# Autodesk Inventor assembly: Swerve-Drivetrain-2
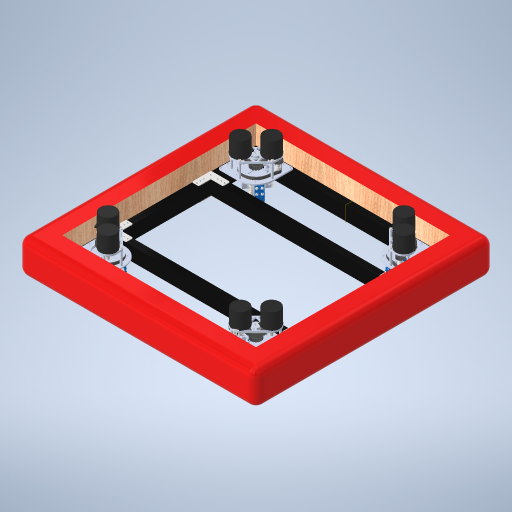
[picture p0: Inventor's stored thumbnail of the model, 512x512]
Saved by Autodesk Inventor 2024.2 (Build 282272000, 272)
## iProperties
Created: 2024-01-06
Part Number: Swerve-Drivetrain-2
Document SubType Name: Assembly
Designer: rohan
Author: rohan
## Documents named in this file (8)
- C:\Users\rohan\OneDrive - Hillsborough County Public Schools\Robotics\FIRST-Robotics-Competition\Crescendo\Minotaur-Crescendo-Robot\Swerve-Drivetrain-2.iam
- C:\Users\rohan\OneDrive - Hillsborough County Public Schools\Robotics\FIRST-Robotics-Competition\Crescendo\Minotaur-Crescendo-Robot\Motion\Swerve-Modules\MK3-Swerve-Module-Falcons-&-Neos.iam
- C:\Users\rohan\OneDrive - Hillsborough County Public Schools\Robotics\FIRST-Robotics-Competition\Crescendo\Minotaur-Crescendo-Robot\Structure\MAXTube\2024-100-002-Front-Back-Extrusions.ipt
- C:\Users\rohan\OneDrive - Hillsborough County Public Schools\Robotics\FIRST-Robotics-Competition\Crescendo\Minotaur-Crescendo-Robot\Structure\MAXTube\2024-100-001-Left-Right-Extrusions.ipt
- C:\Users\rohan\OneDrive - Hillsborough County Public Schools\Robotics\FIRST-Robotics-Competition\Crescendo\Minotaur-Crescendo-Robot\Structure\MAXTube\2024-100-003-Middle-Extrusions.ipt
- C:\Users\rohan\OneDrive - Hillsborough County Public Schools\Robotics\FIRST-Robotics-Competition\Crescendo\Minotaur-Crescendo-Robot\Structure\Gussets\90-Degree-Sharp-Gusset.ipt
- C:\Users\rohan\OneDrive - Hillsborough County Public Schools\Robotics\FIRST-Robotics-Competition\Crescendo\Minotaur-Crescendo-Robot\Structure\Gussets\THRIFYBOT-L-Gusset.ipt
- C:\Users\rohan\OneDrive - Hillsborough County Public Schools\Robotics\FIRST-Robotics-Competition\Crescendo\Minotaur-Crescendo-Robot\Bumpers.ipt
## Components (23 placed, 7 different names)
1. MK3-Swerve-Module-Falcons-&-Neos:1 [sub-assembly] — Mate:10, Mate:56, Mate:57
2. MK3-Swerve-Module-Falcons-&-Neos:2 [sub-assembly] — Mate:7, Mate:9, Mate:20
3. MK3-Swerve-Module-Falcons-&-Neos:3 [sub-assembly] — Mate:4, Mate:16, Tangent:1, Mate:52, Mate:53
4. MK3-Swerve-Module-Falcons-&-Neos:4 [sub-assembly] — Mate:1, Mate:2, Mate:3, Mate:14
5. 2024-100-002-Front-Back-Extrusions:1 — Mate:7, Mate:9, Mate:10, Mate:17, Flush:3, Flush:4, Mate:18, Flush:5, Mate:19, Flush:6, Symmetry:2, Mate:20, Mate:42, Mate:48, Mate:49, Mate:54, Mate:57, Flush:12, Flush:18
6. 2024-100-002-Front-Back-Extrusions:2 — Mate:1, Mate:2, Mate:3, Mate:4, Mate:13, Flush:1, Mate:15, Flush:2, Symmetry:2, Mate:40, Mate:41, Mate:44, Mate:45, Mate:46, Mate:47, Mate:52, Mate:53, Flush:20, Mate:65, Mate:66
7. 2024-100-001-Left-Right-Extrusions:1 — Mate:13, Mate:14, Flush:1, Symmetry:1, Mate:43
8. 2024-100-001-Left-Right-Extrusions:2 — Mate:15, Mate:16, Flush:2, Mate:17, Flush:3, Flush:4, Symmetry:1, Mate:55, Mate:56, Mate:67
9. 2024-100-003-Middle-Extrusions:1 — Mate:19, Flush:6, Symmetry:3, Mate:21, Mate:60, Flush:11, Flush:21
10. 2024-100-003-Middle-Extrusions:2 — Mate:18, Flush:5, Symmetry:3, Mate:21, Mate:61, Flush:13, Mate:64, Flush:19
11. 90-Degree-Sharp-Gusset:1 — Mate:42, Mate:54, Mate:55
12. 90-Degree-Sharp-Gusset:2 — Mate:43, Mate:48, Mate:49
13. 90-Degree-Sharp-Gusset:3 — Mate:41, Mate:44, Mate:45
14. 90-Degree-Sharp-Gusset:4 — Mate:40, Mate:46, Mate:47
15. THRIFYBOT-L-Gusset:1 — Mate:58, Flush:7, Flush:8
16. THRIFYBOT-L-Gusset:2 — Mate:58, Flush:7, Flush:8, Mate:60, Flush:11, Flush:12
17. THRIFYBOT-L-Gusset:3 — Mate:61
18. THRIFYBOT-L-Gusset:4 — Flush:13, Flush:18
19. THRIFYBOT-L-Gusset:5
20. THRIFYBOT-L-Gusset:6 — Mate:65, Flush:21
21. THRIFYBOT-L-Gusset:7
22. THRIFYBOT-L-Gusset:8 — Mate:64, Flush:19, Flush:20
23. Bumpers:1 — Mate:66, Mate:67, Mate:68
## Relationships (68: Mate 43, Flush 21, Symmetry 3, Tangent 1)
- Mate:1: MK3-Swerve-Module-Falcons-&-Neos:4 ↔ 2024-100-002-Front-Back-Extrusions:2
- Mate:2: MK3-Swerve-Module-Falcons-&-Neos:4 ↔ 2024-100-002-Front-Back-Extrusions:2
- Mate:3: MK3-Swerve-Module-Falcons-&-Neos:4 ↔ 2024-100-002-Front-Back-Extrusions:2
- Mate:4: MK3-Swerve-Module-Falcons-&-Neos:3 ↔ 2024-100-002-Front-Back-Extrusions:2
- Mate:7: MK3-Swerve-Module-Falcons-&-Neos:2 ↔ 2024-100-002-Front-Back-Extrusions:1
- Mate:9: MK3-Swerve-Module-Falcons-&-Neos:2 ↔ 2024-100-002-Front-Back-Extrusions:1
- Mate:10: MK3-Swerve-Module-Falcons-&-Neos:1 ↔ 2024-100-002-Front-Back-Extrusions:1
- Mate:13: 2024-100-002-Front-Back-Extrusions:2 ↔ 2024-100-001-Left-Right-Extrusions:1
- Mate:14: MK3-Swerve-Module-Falcons-&-Neos:4 ↔ 2024-100-001-Left-Right-Extrusions:1
- Flush:1: 2024-100-002-Front-Back-Extrusions:2 ↔ 2024-100-001-Left-Right-Extrusions:1
- Mate:15: 2024-100-002-Front-Back-Extrusions:2 ↔ 2024-100-001-Left-Right-Extrusions:2
- Mate:16: MK3-Swerve-Module-Falcons-&-Neos:3 ↔ 2024-100-001-Left-Right-Extrusions:2
- Flush:2: 2024-100-002-Front-Back-Extrusions:2 ↔ 2024-100-001-Left-Right-Extrusions:2
- Mate:17: 2024-100-002-Front-Back-Extrusions:1 ↔ 2024-100-001-Left-Right-Extrusions:2
- Flush:3: 2024-100-002-Front-Back-Extrusions:1 ↔ 2024-100-001-Left-Right-Extrusions:2
- Flush:4: 2024-100-002-Front-Back-Extrusions:1 ↔ 2024-100-001-Left-Right-Extrusions:2
- Mate:18: 2024-100-002-Front-Back-Extrusions:1 ↔ 2024-100-003-Middle-Extrusions:2
- Flush:5: 2024-100-002-Front-Back-Extrusions:1 ↔ 2024-100-003-Middle-Extrusions:2
- Mate:19: 2024-100-002-Front-Back-Extrusions:1 ↔ 2024-100-003-Middle-Extrusions:1
- Flush:6: 2024-100-002-Front-Back-Extrusions:1 ↔ 2024-100-003-Middle-Extrusions:1
- Symmetry:1: 2024-100-001-Left-Right-Extrusions:1 ↔ 2024-100-001-Left-Right-Extrusions:2
- Symmetry:2: 2024-100-002-Front-Back-Extrusions:1 ↔ 2024-100-002-Front-Back-Extrusions:2
- Tangent:1: MK3-Swerve-Module-Falcons-&-Neos:3
- Symmetry:3: 2024-100-003-Middle-Extrusions:1 ↔ 2024-100-003-Middle-Extrusions:2
- Mate:20: MK3-Swerve-Module-Falcons-&-Neos:2 ↔ 2024-100-002-Front-Back-Extrusions:1
- Mate:21 (330.2 mm): 2024-100-003-Middle-Extrusions:1 ↔ 2024-100-003-Middle-Extrusions:2
- Mate:40: 2024-100-002-Front-Back-Extrusions:2 ↔ 90-Degree-Sharp-Gusset:4
- Mate:41: 2024-100-002-Front-Back-Extrusions:2 ↔ 90-Degree-Sharp-Gusset:3
- Mate:42: 2024-100-002-Front-Back-Extrusions:1 ↔ 90-Degree-Sharp-Gusset:1
- Mate:43: 2024-100-001-Left-Right-Extrusions:1 ↔ 90-Degree-Sharp-Gusset:2
- Mate:44: 2024-100-002-Front-Back-Extrusions:2 ↔ 90-Degree-Sharp-Gusset:3
- Mate:45: 2024-100-002-Front-Back-Extrusions:2 ↔ 90-Degree-Sharp-Gusset:3
- Mate:46: 2024-100-002-Front-Back-Extrusions:2 ↔ 90-Degree-Sharp-Gusset:4
- Mate:47: 2024-100-002-Front-Back-Extrusions:2 ↔ 90-Degree-Sharp-Gusset:4
- Mate:48: 2024-100-002-Front-Back-Extrusions:1 ↔ 90-Degree-Sharp-Gusset:2
- Mate:49: 2024-100-002-Front-Back-Extrusions:1 ↔ 90-Degree-Sharp-Gusset:2
- Mate:52: MK3-Swerve-Module-Falcons-&-Neos:3 ↔ 2024-100-002-Front-Back-Extrusions:2
- Mate:53: MK3-Swerve-Module-Falcons-&-Neos:3 ↔ 2024-100-002-Front-Back-Extrusions:2
- Mate:54: 2024-100-002-Front-Back-Extrusions:1 ↔ 90-Degree-Sharp-Gusset:1
- Mate:55: 2024-100-001-Left-Right-Extrusions:2 ↔ 90-Degree-Sharp-Gusset:1
- Mate:56: MK3-Swerve-Module-Falcons-&-Neos:1 ↔ 2024-100-001-Left-Right-Extrusions:2
- Mate:57: MK3-Swerve-Module-Falcons-&-Neos:1 ↔ 2024-100-002-Front-Back-Extrusions:1
- Mate:58 (50.8 mm): THRIFYBOT-L-Gusset:1 ↔ THRIFYBOT-L-Gusset:2
- Flush:7: THRIFYBOT-L-Gusset:1 ↔ THRIFYBOT-L-Gusset:2
- Flush:8: THRIFYBOT-L-Gusset:1 ↔ THRIFYBOT-L-Gusset:2
- [Mate] (50.8 mm): THRIFYBOT-L-Gusset:3 ↔ THRIFYBOT-L-Gusset:4
- [Flush]: THRIFYBOT-L-Gusset:3 ↔ THRIFYBOT-L-Gusset:4
- [Flush]: THRIFYBOT-L-Gusset:3 ↔ THRIFYBOT-L-Gusset:4
- Mate:60: 2024-100-003-Middle-Extrusions:1 ↔ THRIFYBOT-L-Gusset:2
- Flush:11: 2024-100-003-Middle-Extrusions:1 ↔ THRIFYBOT-L-Gusset:2
- Flush:12: 2024-100-002-Front-Back-Extrusions:1 ↔ THRIFYBOT-L-Gusset:2
- Mate:61: 2024-100-003-Middle-Extrusions:2 ↔ THRIFYBOT-L-Gusset:3
- Flush:13: 2024-100-003-Middle-Extrusions:2 ↔ THRIFYBOT-L-Gusset:4
- [Mate] (50.8 mm): THRIFYBOT-L-Gusset:5 ↔ THRIFYBOT-L-Gusset:6
- [Flush]: THRIFYBOT-L-Gusset:5 ↔ THRIFYBOT-L-Gusset:6
- [Flush]: THRIFYBOT-L-Gusset:5 ↔ THRIFYBOT-L-Gusset:6
- [Mate] (50.8 mm): THRIFYBOT-L-Gusset:7 ↔ THRIFYBOT-L-Gusset:8
- [Flush]: THRIFYBOT-L-Gusset:7 ↔ THRIFYBOT-L-Gusset:8
- [Flush]: THRIFYBOT-L-Gusset:7 ↔ THRIFYBOT-L-Gusset:8
- Flush:18: 2024-100-002-Front-Back-Extrusions:1 ↔ THRIFYBOT-L-Gusset:4
- Mate:64: 2024-100-003-Middle-Extrusions:2 ↔ THRIFYBOT-L-Gusset:8
- Flush:19: 2024-100-003-Middle-Extrusions:2 ↔ THRIFYBOT-L-Gusset:8
- Flush:20: 2024-100-002-Front-Back-Extrusions:2 ↔ THRIFYBOT-L-Gusset:8
- Mate:65: 2024-100-002-Front-Back-Extrusions:2 ↔ THRIFYBOT-L-Gusset:6
- Flush:21: 2024-100-003-Middle-Extrusions:1 ↔ THRIFYBOT-L-Gusset:6
- Mate:66: 2024-100-002-Front-Back-Extrusions:2 ↔ Bumpers:1
- Mate:67: 2024-100-001-Left-Right-Extrusions:2 ↔ Bumpers:1
- Mate:68 (38.1 mm): Bumpers:1
## Named parameters: d81_d78 = 50.8 mm, d82_d79 = 0 mm, d83_d80 = 0 mm, d90_d81_d78 = 50.8 mm, d91_d82_d79 = 0 mm, d92_d83_d80 = 0 mm, d93_d90_d81_d78 = 50.8 mm, d94_d91_d82_d79 = 0 mm, d95_d92_d83_d80 = 0 mm
